# Autodesk Inventor assembly: Sestava1
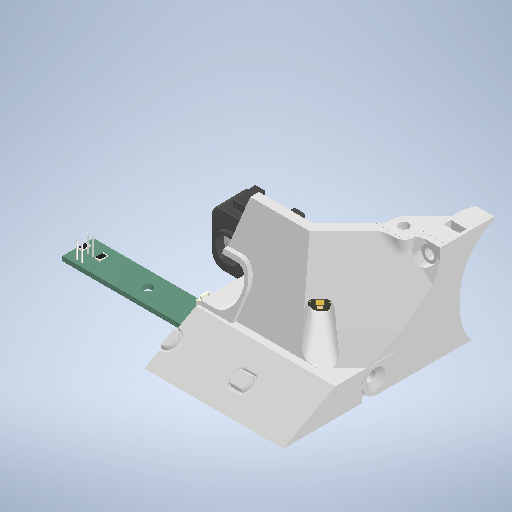
[picture p0: Inventor's stored thumbnail of the model, 512x512]
Saved by Autodesk Inventor 2025.1 (Build 291241000, 241)
## iProperties
Created: 2024-10-19
Part Number: Sestava1
Document SubType Name: Assembly
Designer: Simak
Author: Simak
## Documents named in this file (6)
- C:\Users\jaryj\Desktop\School\Projects\MiniSumo\Sumec-MiniSumo\-3D-\Sestava1.iam
- C:\Users\jaryj\Desktop\School\Projects\MiniSumo\Sumec-MiniSumo\-3D-\3D_printed\body-main.ipt
- C:\Users\jaryj\Desktop\School\Projects\MiniSumo\Sumec-MiniSumo\-3D-\3D_printed\body-front.ipt
- C:\Users\jaryj\Desktop\School\Projects\MiniSumo\Sumec-MiniSumo\-3D-\electronics\pololu-digital-distance-sensor-irs17a.ipt
- C:\Users\jaryj\Desktop\School\Projects\MiniSumo\Sumec-MiniSumo\-3D-\electronics\AssemBeneWake TF-LUNA.ipt
- C:\Users\jaryj\Desktop\School\Projects\MiniSumo\Sumec-MiniSumo\-3D-\electronics\PCBs\QRE MiniBoards\QRE MiniBoards\QRE_MiniBoards_Board.iam
## Components (5 placed, 5 different names)
1. body-main:1 — OPEN, Stejný směr:1, Vložit:1
2. body-front:1 — OPEN, Stejný směr:1, Vložit:1, Stejný směr:2, Proti sobě:2, Proti sobě:3, Proti sobě:4, Úhel:1, Tečnost:1, Vložit:2, Vložit:3
3. pololu-digital-distance-sensor-irs17a:1 — Stejný směr:2, Proti sobě:2, Proti sobě:3
4. AssemBeneWake TF-LUNA:1 — Proti sobě:4, Úhel:1, Tečnost:1
5. QRE_MiniBoards_Board:1 [sub-assembly] — Vložit:2, Vložit:3
## Relationships (11: Mate 4, Insert 3, Flush 2, Angle 1, Tangent 1)
- OPEN [Mate]: body-main:1 ↔ body-front:1
- Stejný směr:1 [Flush]: body-main:1 ↔ body-front:1
- Vložit:1 [Insert]: body-main:1 ↔ body-front:1
- Stejný směr:2 [Flush]: body-front:1 ↔ pololu-digital-distance-sensor-irs17a:1
- Proti sobě:2 [Mate]: body-front:1 ↔ pololu-digital-distance-sensor-irs17a:1
- Proti sobě:3 [Mate]: body-front:1 ↔ pololu-digital-distance-sensor-irs17a:1
- Proti sobě:4 [Mate]: body-front:1 ↔ AssemBeneWake TF-LUNA:1
- Úhel:1 [Angle] (0 deg): body-front:1 ↔ AssemBeneWake TF-LUNA:1
- Tečnost:1 [Tangent] (-0.1 mm): body-front:1 ↔ AssemBeneWake TF-LUNA:1
- Vložit:2 [Insert]: body-front:1 ↔ QRE_MiniBoards_Board:1
- Vložit:3 [Insert]: body-front:1 ↔ QRE_MiniBoards_Board:1
